# Autodesk Inventor assembly: StereoVisionHolder
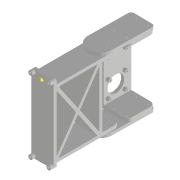
[picture p0: Inventor's stored thumbnail of the model, 180x180]
Saved by Autodesk Inventor 2022 (Build 260153000, 153)
## iProperties
Created: 2022-11-13
Part Number: StereoVisionHolder
Document SubType Name: Assembly
Designer: MVeszpremi
Author: MVeszpremi
## Documents named in this file (4)
- C:\Users\veszp\Dropbox\180DAB CAD\StereoVisionHolder.iam
- C:\Users\veszp\Dropbox\180DAB CAD\StereoVisionHolder.ipt
- C:\Users\veszp\Dropbox\180DAB CAD\StereoVisionHolder_2.ipt
- C:\Users\veszp\Dropbox\180DAB CAD\StereoVisionHolder_3.ipt
## Components (4 placed, 3 different names)
1. StereoVisionHolder:1 — Mate:1, Mate:2, Mate:3, Mate:4
2. StereoVisionHolder_2:1 — Mate:3, Mate:4, Mate:5
3. StereoVisionHolder_2:2 — Mate:1, Mate:2, Mate:5, Mate:6, Mate:7, Mate:8
4. StereoVisionHolder_3:1 — Mate:6, Mate:7, Mate:8
## Relationships (8: Mate 8)
- Mate:1: StereoVisionHolder:1 ↔ StereoVisionHolder_2:2
- Mate:2: StereoVisionHolder:1 ↔ StereoVisionHolder_2:2
- Mate:3: StereoVisionHolder:1 ↔ StereoVisionHolder_2:1
- Mate:4: StereoVisionHolder:1 ↔ StereoVisionHolder_2:1
- Mate:5: StereoVisionHolder_2:1 ↔ StereoVisionHolder_2:2
- Mate:6: StereoVisionHolder_2:2 ↔ StereoVisionHolder_3:1
- Mate:7: StereoVisionHolder_2:2 ↔ StereoVisionHolder_3:1
- Mate:8: StereoVisionHolder_2:2 ↔ StereoVisionHolder_3:1
